# Autodesk Inventor assembly: HS 36T Gear, No Insert_MIR
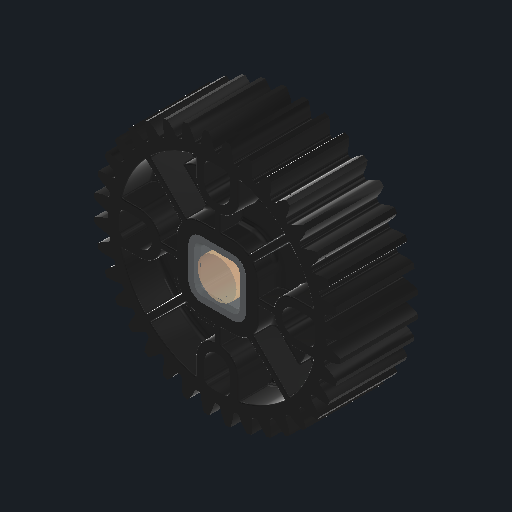
[picture p0: Inventor's stored thumbnail of the model, 512x512]
Saved by Autodesk Inventor 2024 (Build 280153000, 153)
## iProperties
Created: 2022-08-02
Part Number: HS 36T Gear, No Insert_MIR
Document SubType Name: Assembly
Designer: avere
Author: ylu12
## Documents named in this file (2)
- C:\Users\avere\Documents\rbp_cad\zoomba_v0.3\chassis\mirrored_parts\HS 36T Gear, No Insert_MIR.iam
- C:\Users\avere\Documents\rbp_cad\zoomba_v0.3\chassis\mirrored_parts\HS 36T Gear, No Insert_MIR.ipt
## Components (1 placed, 1 different names)
1. HS 36T Gear, No Insert_MIR:1 — Mate:10, Mate:9, Flush:5
## Relationships (3: Mate 2, Flush 1)
- Mate:10: HS 36T Gear, No Insert_MIR:1
- Mate:9: HS 36T Gear, No Insert_MIR:1
- Flush:5: HS 36T Gear, No Insert_MIR:1
